# Autodesk Inventor assembly: A2017_T3_02
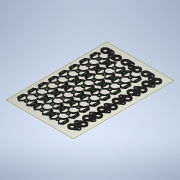
[picture p0: Inventor's stored thumbnail of the model, 180x180]
Saved by Autodesk Inventor 2022 (Build 260153000, 153)
## iProperties
Created: 2022-09-28
Part Number: A2017_T3_02
Document SubType Name: Assembly
Designer: Masato
Author: Masato
## Documents named in this file (4)
- C:\Users\ヨコオリク\Documents\CITBrains\SUSTAINA-OP\Cam\A2017_T3\A2017_T3_02.iam
- C:\Users\ヨコオリク\Documents\CITBrains\SUSTAINA-OP\Cam\DisposableBoard.ipt
- C:\Users\ヨコオリク\Documents\CITBrains\SUSTAINA-OP\LowerBody\Slider_crank\Slider_crank_horn.ipt
- C:\Users\ヨコオリク\Documents\CITBrains\SUSTAINA-OP\LowerBody\Leg_joint\Leg_joint_roll_frame.ipt
## Components (42 placed, 3 different names)
1. DisposableBoard:1 — フラッシュ:1, フラッシュ:2, フラッシュ:3, フラッシュ:4, Tangent:1, Flush:5, Flush:6, Tangent:2, 正接:3, 正接:4, 正接:5
2. Slider_crank_horn:17 — メイト:10, メイト:11, 正接:5
3. Leg_joint_roll_frame:2 — Tangent:1, Flush:5, Mate:5
4. Leg_joint_roll_frame:3
5. Leg_joint_roll_frame:4
6. Leg_joint_roll_frame:5
7. Leg_joint_roll_frame:6
8. Leg_joint_roll_frame:7
9. Leg_joint_roll_frame:8
10. Leg_joint_roll_frame:9
11. Leg_joint_roll_frame:10
12. Leg_joint_roll_frame:11
13. Leg_joint_roll_frame:12
14. Leg_joint_roll_frame:13
15. Leg_joint_roll_frame:14
16. Leg_joint_roll_frame:15
17. Leg_joint_roll_frame:16
18. Leg_joint_roll_frame:17
19. Leg_joint_roll_frame:18
20. Leg_joint_roll_frame:19
21. Leg_joint_roll_frame:20
22. Leg_joint_roll_frame:21
23. Leg_joint_roll_frame:22
24. Leg_joint_roll_frame:23 — Mate:4
25. Leg_joint_roll_frame:24
26. Leg_joint_roll_frame:25
27. Slider_crank_horn:2 — Mate:1, Mate:2, Mate:4
28. Slider_crank_horn:1 — Flush:6, Mate:1, Mate:3, Tangent:2
29. Slider_crank_horn:3
30. Slider_crank_horn:4
31. Slider_crank_horn:5 — メイト:7
32. Slider_crank_horn:6
33. Slider_crank_horn:7 — メイト:6, メイト:7, 正接:3, メイト:9
34. Slider_crank_horn:8 — メイト:8, メイト:9, 正接:4
35. Slider_crank_horn:9
36. Slider_crank_horn:10
37. Slider_crank_horn:11
38. Slider_crank_horn:12
39. Slider_crank_horn:13
40. Slider_crank_horn:14
41. Slider_crank_horn:15
42. Slider_crank_horn:16 — メイト:11
## Component patterns: (24 elements, first: Leg_joint_roll_frame:2), (3 elements, first: Slider_crank_horn:2 + Slider_crank_horn:1), (5 elements, first: Slider_crank_horn:7 + Slider_crank_horn:8)
## Relationships (22: Mate 11, Flush 6, Tangent 5)
- フラッシュ:1 [Flush]: DisposableBoard:1
- フラッシュ:2 [Flush]: DisposableBoard:1
- フラッシュ:3 [Flush]: DisposableBoard:1
- フラッシュ:4 [Flush]: DisposableBoard:1
- Tangent:1 (2 mm): DisposableBoard:1 ↔ Leg_joint_roll_frame:2
- Flush:5 (-2 mm): DisposableBoard:1 ↔ Leg_joint_roll_frame:2
- Flush:6 (-2.1 mm): DisposableBoard:1 ↔ Slider_crank_horn:1
- Mate:1 (2.1 mm): Slider_crank_horn:2 ↔ Slider_crank_horn:1
- Mate:2: Slider_crank_horn:2
- Mate:3: Slider_crank_horn:1
- Tangent:2 (2 mm): DisposableBoard:1 ↔ Slider_crank_horn:1
- Mate:4 (2.1 mm): Leg_joint_roll_frame:23 ↔ Slider_crank_horn:2
- Mate:5: Leg_joint_roll_frame:2
- メイト:6 [Mate]: Slider_crank_horn:7
- メイト:7 [Mate] (2.5 mm): Slider_crank_horn:5 ↔ Slider_crank_horn:7
- 正接:3 [Tangent] (2 mm): DisposableBoard:1 ↔ Slider_crank_horn:7
- メイト:8 [Mate]: Slider_crank_horn:8
- メイト:9 [Mate] (2.5 mm): Slider_crank_horn:7 ↔ Slider_crank_horn:8
- 正接:4 [Tangent] (2 mm): DisposableBoard:1 ↔ Slider_crank_horn:8
- メイト:10 [Mate]: Slider_crank_horn:17
- メイト:11 [Mate] (2.5 mm): Slider_crank_horn:17 ↔ Slider_crank_horn:16
- 正接:5 [Tangent] (2 mm): DisposableBoard:1 ↔ Slider_crank_horn:17
